# Autodesk Inventor assembly: E8T-X-250-S-D-D-X
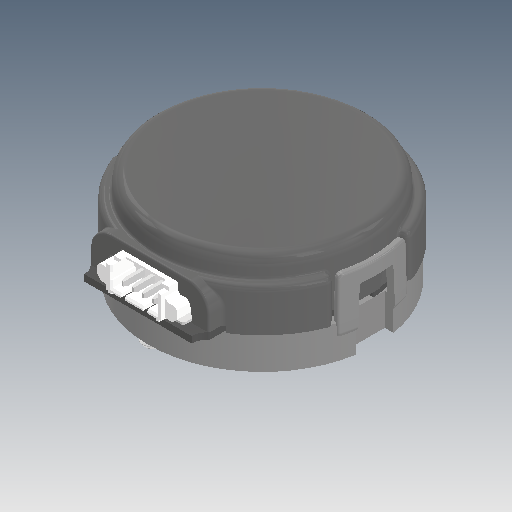
[picture p0: Inventor's stored thumbnail of the model, 512x512]
Saved by Autodesk Inventor 2020 (Build 240168000, 168)
## iProperties
Created: 2019-11-15
Part Number: E8T-X-250-S-D-D-X
Document SubType Name: Assembly
Designer: ball
Author: ball
## Documents named in this file (3)
- C:\FTC\FTC8863CAD\2019 Robot\Odoemetry module\E8T-X-250-S-D-D-X.iam
- C:\FTC\FTC8863CAD\2019 Robot\Odoemetry module\E8T-X-250-S-D-D-X.ipt
- C:\FTC\FTC8863CAD\2019 Robot\Odoemetry module\92095A459_18-8 SS BUTTON-HEAD SOCKET CAP SCREW.ipt
## Components (3 placed, 2 different names)
1. E8T-X-250-S-D-D-X:1 — Mate:1, Mate:2, Mate:3, Mate:4
2. 92095A459_18-8 SS BUTTON-HEAD SOCKET CAP SCREW:1 — Mate:1, Mate:2
3. 92095A459_18-8 SS BUTTON-HEAD SOCKET CAP SCREW:2 — Mate:3, Mate:4
## Relationships (4: Mate 4)
- Mate:1: E8T-X-250-S-D-D-X:1 ↔ 92095A459_18-8 SS BUTTON-HEAD SOCKET CAP SCREW:1
- Mate:2: E8T-X-250-S-D-D-X:1 ↔ 92095A459_18-8 SS BUTTON-HEAD SOCKET CAP SCREW:1
- Mate:3: E8T-X-250-S-D-D-X:1 ↔ 92095A459_18-8 SS BUTTON-HEAD SOCKET CAP SCREW:2
- Mate:4: E8T-X-250-S-D-D-X:1 ↔ 92095A459_18-8 SS BUTTON-HEAD SOCKET CAP SCREW:2
